# Autodesk Inventor assembly: Vert - 1in
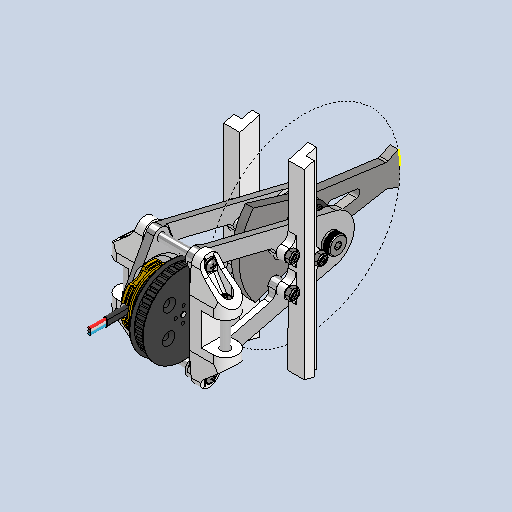
[picture p0: Inventor's stored thumbnail of the model, 512x512]
Saved by Autodesk Inventor 2023.2 (Build 272271000, 271)
## iProperties
Created: 2023-07-17
Part Number: Vert - 1in
Document SubType Name: Assembly
Designer: Nathan Cai
Mass: 651.349 g
Surface Area: 1336.54 cm^2
Volume: 224.034 cm^3
Density: 2.90737 g/cm^3
Author: Nathan Cai
## Documents named in this file (21)
- E:\Documents\Inventor\Law - V2.0\Vert - Cheap\Vert - Cheap.iam
- E:\Documents\Inventor\Law - V2.0\Vert - 1in\6-32 x 5-8.ipt
- E:\Documents\Inventor\Law - V2.0\Vert - 1in\6-32 Nylock.ipt
- E:\Documents\Inventor\Content Center Files\R2023\en-US\ANSI B18.22.1\ANSI B18.22.1 - No. 6 - Type A.ipt
- E:\Documents\Inventor\Content Center Files\R2023\en-US\ANSI B18.6.3(27)\ANSI B18.6.3 - 6-32 UNC - 0.375(11).ipt
- E:\Documents\Inventor\Content Center Files\R2023\en-US\ANSI B18.6.3(27)\ANSI B18.6.3 - 6-32 UNC - 0.75(11).ipt
- E:\Documents\Inventor\Law - V2.0\Vert - Cheap\FEICHAO BE4108 380KV\FEICHAO BE4108 380KV.iam
- E:\Documents\Inventor\Law - V2.0\Vert - Cheap\Blade (Bar 3).ipt
- E:\Documents\Inventor\Law - V2.0\Vert - Cheap\Upright - Motor.ipt
- E:\Documents\Inventor\Law - V2.0\Vert - Cheap\Upright - Blank.ipt
- E:\Documents\Inventor\Law - V2.0\Vert - Cheap\Leg.ipt
- E:\Documents\Inventor\Law - V2.0\Vert - Cheap\91259A628_Alloy Steel Shoulder Screw.ipt
- E:\Documents\Inventor\Law - V2.0\Vert - Cheap\90630A121_High-Strength Steel Nylon-Insert Locknut.ipt
- E:\Documents\Inventor\Law - V2.0\Vert - Cheap\XL Pulley 18T .25in Wd.ipt
- E:\Documents\Inventor\Law - V2.0\Vert - Cheap\XL Pulley 36T .375in Wd.ipt
- E:\Documents\Inventor\Law - V2.0\Vert - Cheap\Spacer 3-8x .125.ipt
- E:\Documents\Inventor\Law - V2.0\Vert - Cheap\Needle Bearings.ipt
- E:\Documents\Inventor\Law - V2.0\Vert - Cheap\5905K497_Needle-Roller Bearing (1).ipt
- E:\Documents\Inventor\Law - V2.0\Vert - Cheap\Standoff 1.5in.ipt
- E:\Documents\Inventor\Law - V2.0\Vert - Cheap\Bracket - Clear.ipt
- E:\Documents\Inventor\Law - V2.0\Vert - Cheap\Standoff 1in.ipt
## Components (49 placed, 20 different names)
1. FEICHAO BE4108 380KV:2 [sub-assembly] — Mate:11
2. Blade (Bar 3):2 — Mate:37
3. Upright - Motor:2 — Mate:11, Mate:24, Mate:103, Mate:104, Mate:106, Mate:108, Mate:109, Mate:110, Mate:111
4. Upright - Blank:2 — Mate:23, Mate:103, Mate:104
5. Leg:3
6. Leg:4
7. 91259A628_Alloy Steel Shoulder Screw:2 — Mate:23, Mate:105, Mate:106
8. 90630A121_High-Strength Steel Nylon-Insert Locknut:2 — Mate:24
9. XL Pulley 18T .25in Wd:2 — Mate:37, Mate:40, Flush:2, Flush:3, Mate:105, Mate:107
10. XL Pulley 36T .375in Wd:2 — Flush:3
11. Spacer 3-8x .125:2 — Mate:107
12. Needle Bearings:3
13. Needle Bearings:4
14. 5905K497_Needle-Roller Bearing (1):3
15. 5905K497_Needle-Roller Bearing (1):4 — Mate:40, Flush:2
16. Standoff 1in:1 — Mate:108, Mate:109
17. Standoff 1in:2 — Mate:110, Mate:111
18. 6-32 x 5-8:1 — Mate:55
19. 6-32 x 5-8:2 — Mate:56
20. 6-32 x 5-8:3 — Mate:57
21. 6-32 x 5-8:4 — Mate:67
22. 6-32 x 5-8:5 — Mate:68
23. 6-32 x 5-8:6 — Mate:69
24. 6-32 Nylock:1 — Mate:67
25. 6-32 Nylock:2 — Mate:69
26. 6-32 Nylock:3 — Mate:68
27. 6-32 Nylock:4 — Mate:56
28. 6-32 Nylock:5 — Mate:57
29. 6-32 Nylock:6 — Mate:55
30. Cross Recessed Truss Head Machine Screw - Type I - Inch No. 6 - 32 - 3/4:5 — Insert:10
31. Plain Washer (Inch) No. 6 - Type A:8 — Mate:114, Mate:115, Insert:10
32. Cross Recessed Truss Head Machine Screw - Type I - Inch No. 6 - 32 - 3/4:1 — Insert:9
33. Plain Washer (Inch) No. 6 - Type A:7 — Mate:112, Mate:113, Insert:9
34. Bracket - Clear:3 — Mate:112, Mate:113, Mate:114, Mate:115
35. Standoff 1.5in:4
36. Plain Washer (Inch) No. 6 - Type A:1 — Insert:1
37. Cross Recessed Truss Head Machine Screw - Type I - Inch No. 6 - 32 - 3/8:1 — Insert:1
38. Plain Washer (Inch) No. 6 - Type A:2 — Insert:2
39. Cross Recessed Truss Head Machine Screw - Type I - Inch No. 6 - 32 - 3/8:2 — Insert:2
40. Standoff 1.5in:3
41. Bracket - Clear:2
42. Plain Washer (Inch) No. 6 - Type A:3 — Insert:5
43. Cross Recessed Truss Head Machine Screw - Type I - Inch No. 6 - 32 - 3/8:3 — Insert:5
44. Plain Washer (Inch) No. 6 - Type A:4 — Insert:6
45. Cross Recessed Truss Head Machine Screw - Type I - Inch No. 6 - 32 - 3/8:4 — Insert:6
46. Plain Washer (Inch) No. 6 - Type A:5 — Insert:7
47. Cross Recessed Truss Head Machine Screw - Type I - Inch No. 6 - 32 - 3/4:3 — Insert:7
48. Plain Washer (Inch) No. 6 - Type A:6 — Insert:8
49. Cross Recessed Truss Head Machine Screw - Type I - Inch No. 6 - 32 - 3/4:4 — Insert:8
## Relationships (98: Mate 84, Insert 8, Flush 6)
- [Mate]: FEICHAO BE4108 380KV:2 ↔ Upright - Motor:2
- [Mate]: FEICHAO BE4108 380KV:2 ↔ Upright - Motor:2
- [Mate]: Blade (Bar 3):2 ↔ Upright - Motor:2
- Mate:11: FEICHAO BE4108 380KV:2 ↔ Upright - Motor:2
- [Mate]: Upright - Motor:2 ↔ Leg:3
- [Mate]: Upright - Motor:2 ↔ Leg:3
- [Mate]: Upright - Motor:2 ↔ Leg:3
- [Mate]: Upright - Blank:2 ↔ Leg:4
- [Mate]: Upright - Blank:2 ↔ Leg:4
- [Mate]: Upright - Blank:2 ↔ Leg:4
- [Mate]: Upright - Blank:2 ↔ 91259A628_Alloy Steel Shoulder Screw:2
- Mate:23: Upright - Blank:2 ↔ 91259A628_Alloy Steel Shoulder Screw:2
- Mate:24: Upright - Motor:2 ↔ 90630A121_High-Strength Steel Nylon-Insert Locknut:2
- [Mate]: 91259A628_Alloy Steel Shoulder Screw:2 ↔ 90630A121_High-Strength Steel Nylon-Insert Locknut:2
- [Mate]: Blade (Bar 3):2 ↔ Spacer 3-8x .125:2
- [Mate]: Blade (Bar 3):2 ↔ Spacer 3-8x .125:2
- [Mate]: 91259A628_Alloy Steel Shoulder Screw:2 ↔ Needle Bearings:3
- [Mate]: Upright - Motor:2 ↔ Needle Bearings:3
- [Mate]: 91259A628_Alloy Steel Shoulder Screw:2 ↔ Needle Bearings:4
- [Mate]: Upright - Blank:2 ↔ Needle Bearings:4
- Mate:37: Blade (Bar 3):2 ↔ XL Pulley 18T .25in Wd:2
- [Mate]: Blade (Bar 3):2 ↔ Spacer 3-8x .125:2
- Mate:40: XL Pulley 18T .25in Wd:2 ↔ 5905K497_Needle-Roller Bearing (1):4
- [Mate]: Blade (Bar 3):2 ↔ 5905K497_Needle-Roller Bearing (1):3
- [Flush]: Spacer 3-8x .125:2 ↔ 5905K497_Needle-Roller Bearing (1):3
- Flush:2: XL Pulley 18T .25in Wd:2 ↔ 5905K497_Needle-Roller Bearing (1):4
- [Mate]: Spacer 3-8x .125:2 ↔ Needle Bearings:3
- Flush:3: XL Pulley 18T .25in Wd:2 ↔ XL Pulley 36T .375in Wd:2
- [Mate]: FEICHAO BE4108 380KV:2 ↔ XL Pulley 36T .375in Wd:2
- [Mate]: FEICHAO BE4108 380KV:2 ↔ XL Pulley 36T .375in Wd:2
- [Mate]: Upright - Blank:2 ↔ 6-32 x 5-8:3
- [Mate]: Upright - Blank:2 ↔ 6-32 x 5-8:2
- [Mate]: Upright - Blank:2 ↔ 6-32 x 5-8:1
- [Mate]: Upright - Blank:2 ↔ 6-32 x 5-8:2
- [Mate]: Upright - Blank:2 ↔ 6-32 x 5-8:1
- [Mate]: Upright - Blank:2 ↔ 6-32 x 5-8:1
- [Mate]: Upright - Blank:2 ↔ 6-32 x 5-8:3
- [Mate]: Leg:4 ↔ 6-32 Nylock:4
- [Mate]: Leg:4 ↔ 6-32 Nylock:5
- [Mate]: Leg:4 ↔ 6-32 Nylock:6
- Mate:55: 6-32 x 5-8:1 ↔ 6-32 Nylock:6
- Mate:56: 6-32 x 5-8:2 ↔ 6-32 Nylock:4
- Mate:57: 6-32 x 5-8:3 ↔ 6-32 Nylock:5
- [Mate]: Upright - Motor:2 ↔ 6-32 x 5-8:5
- [Mate]: Upright - Motor:2 ↔ 6-32 x 5-8:4
- [Mate]: Upright - Motor:2 ↔ 6-32 x 5-8:6
- [Mate]: Upright - Motor:2 ↔ 6-32 x 5-8:5
- [Mate]: Upright - Motor:2 ↔ 6-32 x 5-8:6
- [Mate]: Upright - Motor:2 ↔ 6-32 x 5-8:4
- [Mate]: Leg:3 ↔ 6-32 Nylock:1
- [Mate]: Leg:3 ↔ 6-32 Nylock:3
- [Mate]: Leg:3 ↔ 6-32 Nylock:2
- Mate:67: 6-32 x 5-8:4 ↔ 6-32 Nylock:1
- Mate:68: 6-32 x 5-8:5 ↔ 6-32 Nylock:3
- Mate:69: 6-32 x 5-8:6 ↔ 6-32 Nylock:2
- [Mate]: Upright - Motor:2 ↔ Bracket - Clear:3
- [Mate]: Upright - Motor:2 ↔ Bracket - Clear:3
- [Mate]: Bracket - Clear:3 ↔ Standoff 1.5in:4
- [Flush]: Bracket - Clear:3 ↔ Standoff 1.5in:4
- [Mate]: Standoff 1.5in:4 ↔ Plain Washer (Inch) No. 6 - Type A:1
- [Mate]: Standoff 1.5in:4 ↔ Plain Washer (Inch) No. 6 - Type A:1
- Insert:1: Plain Washer (Inch) No. 6 - Type A:1 ↔ Cross Recessed Truss Head Machine Screw - Type I - Inch No. 6 - 32 - 3/8:1
- [Mate]: Standoff 1.5in:4 ↔ Plain Washer (Inch) No. 6 - Type A:2
- [Mate]: Standoff 1.5in:4 ↔ Plain Washer (Inch) No. 6 - Type A:2
- Insert:2: Plain Washer (Inch) No. 6 - Type A:2 ↔ Cross Recessed Truss Head Machine Screw - Type I - Inch No. 6 - 32 - 3/8:2
- [Mate]: Standoff 1.5in:3 ↔ Bracket - Clear:2
- [Flush]: Standoff 1.5in:3 ↔ Bracket - Clear:2
- [Mate]: Standoff 1.5in:3 ↔ Plain Washer (Inch) No. 6 - Type A:3
- [Mate]: Standoff 1.5in:3 ↔ Plain Washer (Inch) No. 6 - Type A:3
- Insert:5: Plain Washer (Inch) No. 6 - Type A:3 ↔ Cross Recessed Truss Head Machine Screw - Type I - Inch No. 6 - 32 - 3/8:3
- [Mate]: Standoff 1.5in:3 ↔ Plain Washer (Inch) No. 6 - Type A:4
- [Mate]: Standoff 1.5in:3 ↔ Plain Washer (Inch) No. 6 - Type A:4
- Insert:6: Plain Washer (Inch) No. 6 - Type A:4 ↔ Cross Recessed Truss Head Machine Screw - Type I - Inch No. 6 - 32 - 3/8:4
- [Mate]: Bracket - Clear:2 ↔ Plain Washer (Inch) No. 6 - Type A:5
- [Mate]: Bracket - Clear:2 ↔ Plain Washer (Inch) No. 6 - Type A:5
- [Mate]: Bracket - Clear:2 ↔ Plain Washer (Inch) No. 6 - Type A:6
- [Mate]: Bracket - Clear:2 ↔ Plain Washer (Inch) No. 6 - Type A:6
- Insert:7: Plain Washer (Inch) No. 6 - Type A:5 ↔ Cross Recessed Truss Head Machine Screw - Type I - Inch No. 6 - 32 - 3/4:3
- Insert:8: Plain Washer (Inch) No. 6 - Type A:6 ↔ Cross Recessed Truss Head Machine Screw - Type I - Inch No. 6 - 32 - 3/4:4
- [Flush]: Bracket - Clear:3 ↔ Bracket - Clear:2
- [Mate]: Bracket - Clear:3 ↔ Bracket - Clear:2
- [Mate]: Upright - Blank:2 ↔ Bracket - Clear:2
- [Mate]: Upright - Motor:2 ↔ Bracket - Clear:3
- Mate:103: Upright - Motor:2 ↔ Upright - Blank:2
- Mate:104 (25.4 mm): Upright - Motor:2 ↔ Upright - Blank:2
- Mate:105: 91259A628_Alloy Steel Shoulder Screw:2 ↔ XL Pulley 18T .25in Wd:2
- Mate:106: Upright - Motor:2 ↔ 91259A628_Alloy Steel Shoulder Screw:2
- Mate:107: XL Pulley 18T .25in Wd:2 ↔ Spacer 3-8x .125:2
- Mate:108: Upright - Motor:2 ↔ Standoff 1in:1
- Mate:109: Upright - Motor:2 ↔ Standoff 1in:1
- Mate:110: Upright - Motor:2 ↔ Standoff 1in:2
- Mate:111: Upright - Motor:2 ↔ Standoff 1in:2
- Mate:112: Plain Washer (Inch) No. 6 - Type A:7 ↔ Bracket - Clear:3
- Mate:113: Plain Washer (Inch) No. 6 - Type A:7 ↔ Bracket - Clear:3
- Mate:114: Plain Washer (Inch) No. 6 - Type A:8 ↔ Bracket - Clear:3
- Mate:115: Plain Washer (Inch) No. 6 - Type A:8 ↔ Bracket - Clear:3
- Insert:9: Cross Recessed Truss Head Machine Screw - Type I - Inch No. 6 - 32 - 3/4:1 ↔ Plain Washer (Inch) No. 6 - Type A:7
- Insert:10: Cross Recessed Truss Head Machine Screw - Type I - Inch No. 6 - 32 - 3/4:5 ↔ Plain Washer (Inch) No. 6 - Type A:8
